# Autodesk Inventor assembly: Assembly1
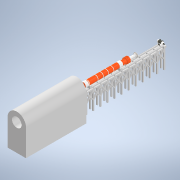
[picture p0: Inventor's stored thumbnail of the model, 180x180]
Saved by Autodesk Inventor 2021 (Build 250183000, 183)
## iProperties
Created: 2021-04-19
Part Number: Assembly1
Document SubType Name: Assembly
Designer: miw14
Author: miw14
## Documents named in this file (11)
- C:\Users\miw14\Desktop\spring2021\mechanics sys\project\Assembly1.iam
- C:\Users\miw14\Desktop\spring2021\mechanics sys\project\rail.ipt
- C:\Users\miw14\Desktop\spring2021\mechanics sys\project\rail part.ipt
- C:\Users\miw14\Desktop\spring2021\mechanics sys\project\City Machine Technologies-98972-RGALA_98972-CGTLA.ipt
- C:\Users\miw14\Desktop\spring2021\mechanics sys\project\City Machine Technologies-98972-RGALA_98972-RGXLA.ipt
- C:\Users\miw14\Desktop\spring2021\mechanics sys\project\City Machine Technologies-98972-RGALA_98972-CGELA.ipt
- C:\Users\miw14\Desktop\spring2021\mechanics sys\project\seat.ipt
- C:\Users\miw14\Desktop\spring2021\mechanics sys\project\roller placemnet.ipt
- C:\Users\miw14\Desktop\spring2021\mechanics sys\project\platform part.ipt
- C:\Users\miw14\Desktop\spring2021\mechanics sys\project\GH50 winch.ipt
- C:\Users\miw14\Desktop\spring2021\mechanics sys\project\stator unit.ipt
## Components (32 placed, 10 different names)
1. City Machine Technologies-98972-RGALA_98972-CGTLA:1 — Insert:1
2. City Machine Technologies-98972-RGALA_98972-RGXLA:1 — Insert:1, Insert:2, Insert:3, Insert:4
3. City Machine Technologies-98972-RGALA_98972-CGELA:1 — Insert:2
4. seat:1 — Mate:5, Mate:6, Mate:7, Mate:8, Mate:9, Mate:10, Insert:3
5. roller placemnet:1 — Mate:5, Mate:6, Mate:7, Mate:18, Mate:20
6. roller placemnet:2 — Mate:8, Mate:9, Mate:10, Mate:17
7. seat:3 — Insert:4, Mate:21
8. roller placemnet:5
9. roller placemnet:6 — Mate:19
10. platform part:1 — Mate:22, Flush:9, Flush:10, Mate:26, Mate:27, Flush:18
11. platform part:2 — Flush:11, Mate:23, Flush:12, Mate:24, Flush:13, Flush:15, Flush:17
12. GH50 winch:1 — Mate:25, Flush:14, Flush:16
13. seat:4 — Mate:24, Flush:13, Mate:25, Flush:15, Flush:16
14. stator unit:1 — Flush:17, Mate:26, Mate:27, Flush:18
15. rail:2 — Mate:3, Flush:7, Flush:8, Mate:18, Mate:20
16. rail:1 — Mate:4, Flush:5, Flush:6, Mate:17, Mate:21
17. rail:3 — Mate:19
18. rail:4
19. rail:5
20. rail:6 — Flush:14
21. rail part:3 — Mate:3, Mate:4, Flush:5, Flush:6, Flush:7, Flush:8, Mate:22, Flush:9, Flush:10, Flush:11, Mate:23, Flush:12
22. rail part:4
23. rail part:5
24. rail part:6
25. rail part:7
26. rail part:8
27. rail part:9
28. rail part:10
29. rail part:11
30. rail part:12
31. rail part:13
32. rail part:14
## Component patterns: (3 elements, first: rail:2 + rail:1), (4 elements, first: rail part:3), Component Pattern 1:2 (4 elements), Component Pattern 1:3 (4 elements)
## Relationships (43: Mate 25, Flush 14, Insert 4)
- Mate:3: rail:2 ↔ rail part:3
- Mate:4: rail:1 ↔ rail part:3
- Flush:5: rail:1 ↔ rail part:3
- Flush:6: rail:1 ↔ rail part:3
- Flush:7: rail:2 ↔ rail part:3
- Flush:8: rail:2 ↔ rail part:3
- Insert:1: City Machine Technologies-98972-RGALA_98972-CGTLA:1 ↔ City Machine Technologies-98972-RGALA_98972-RGXLA:1
- Insert:2: City Machine Technologies-98972-RGALA_98972-RGXLA:1 ↔ City Machine Technologies-98972-RGALA_98972-CGELA:1
- Mate:5: seat:1 ↔ roller placemnet:1
- Mate:6: seat:1 ↔ roller placemnet:1
- Mate:7: seat:1 ↔ roller placemnet:1
- Mate:8: seat:1 ↔ roller placemnet:2
- Mate:9: seat:1 ↔ roller placemnet:2
- Mate:10: seat:1 ↔ roller placemnet:2
- [Mate]: seat:3 ↔ roller placemnet:5
- [Mate]: seat:3 ↔ roller placemnet:5
- [Mate]: seat:3 ↔ roller placemnet:5
- [Mate]: seat:3 ↔ roller placemnet:6
- [Mate]: seat:3 ↔ roller placemnet:6
- [Mate]: seat:3 ↔ roller placemnet:6
- Insert:3: City Machine Technologies-98972-RGALA_98972-RGXLA:1 ↔ seat:1
- Insert:4: City Machine Technologies-98972-RGALA_98972-RGXLA:1 ↔ seat:3
- Mate:17: roller placemnet:2 ↔ rail:1
- Mate:18: roller placemnet:1 ↔ rail:2
- Mate:19: roller placemnet:6 ↔ rail:3
- Mate:20: roller placemnet:1 ↔ rail:2
- Mate:21: seat:3 ↔ rail:1
- Mate:22: platform part:1 ↔ rail part:3
- Flush:9: platform part:1 ↔ rail part:3
- Flush:10: platform part:1 ↔ rail part:3
- Flush:11: platform part:2 ↔ rail part:3
- Mate:23: platform part:2 ↔ rail part:3
- Flush:12: platform part:2 ↔ rail part:3
- Mate:24: platform part:2 ↔ seat:4
- Flush:13: platform part:2 ↔ seat:4
- Mate:25: GH50 winch:1 ↔ seat:4
- Flush:14: GH50 winch:1 ↔ rail:6
- Flush:15: platform part:2 ↔ seat:4
- Flush:16: GH50 winch:1 ↔ seat:4
- Flush:17: platform part:2 ↔ stator unit:1
- Mate:26: platform part:1 ↔ stator unit:1
- Mate:27: platform part:1 ↔ stator unit:1
- Flush:18: platform part:1 ↔ stator unit:1
## Named parameters: d28_d22 = 0 mm, d29_d23 = 0 mm, d30_d24 = 0 mm, d31_d25 = 0 mm, d32_d26 = 0 mm, d33_d27 = 0 mm
